# Autodesk Inventor assembly: Stepper Motor NEMA 17
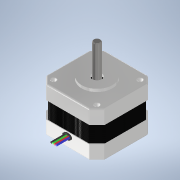
[picture p0: Inventor's stored thumbnail of the model, 180x180]
Saved by Autodesk Inventor 2022 (Build 260153000, 153)
## iProperties
Created: 2021-06-25
Part Number: Stepper Motor NEMA 17
Document SubType Name: Assembly
Designer: Work
Author: Work
## Documents named in this file (4)
- C:\Users\John\Desktop\P3 Bracket Files\Given Files\3. Rotary Actuator Assembly\Stepper Motor NEMA 17.iam
- C:\Users\John\Desktop\P3 Bracket Files\Given Files\3. Rotary Actuator Assembly\Piece1.ipt
- C:\Users\John\Desktop\P3 Bracket Files\Given Files\3. Rotary Actuator Assembly\Piece2.ipt
- C:\Users\John\Desktop\P3 Bracket Files\Given Files\Stepper Updated\Stepper Motor Shaft.ipt
## Components (3 placed, 3 different names)
1. Piece1:1 — Mate:1, Flush:1, Flush:2, Insert:1
2. Piece2:1 — Mate:1, Flush:1, Flush:2
3. Stepper Motor Shaft:1 — Insert:1
## Relationships (4: Flush 2, Mate 1, Insert 1)
- Mate:1: Piece1:1 ↔ Piece2:1
- Flush:1: Piece1:1 ↔ Piece2:1
- Flush:2: Piece1:1 ↔ Piece2:1
- Insert:1: Piece1:1 ↔ Stepper Motor Shaft:1
